# Autodesk Inventor assembly: ballShooterV03
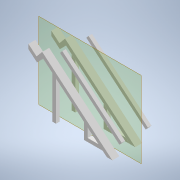
[picture p0: Inventor's stored thumbnail of the model, 180x180]
Saved by Autodesk Inventor 2020.2 (Build 242310000, 310)
## iProperties
Created: 2020-02-22
Part Number: ballShooterV03
Document SubType Name: Assembly
Designer: robst
Author: robst
## Documents named in this file (3)
- C:\git\CAD-Development\robSteele\2020LongRobotBase\ballShooterV03.iam
- C:\git\CAD-Development\robSteele\2020LongRobotBase\rightHalfOfFrameV03.iam
- C:\git\CAD-Development\robSteele\2020LongRobotBase\rightHalfOfFrameV03_MIR.iam
## Components (2 placed, 2 different names)
1. rightHalfOfFrameV03:1 [sub-assembly] — Flush:1
2. rightHalfOfFrameV03_MIR:1 [sub-assembly] — Mate:1
## Relationships (2: Flush 1, Mate 1)
- Flush:1 (57.15 mm): rightHalfOfFrameV03:1
- Mate:1 (57.15 mm): rightHalfOfFrameV03_MIR:1
